# Autodesk Inventor assembly: PIVOT_FRAMING
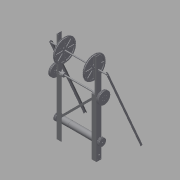
[picture p0: Inventor's stored thumbnail of the model, 180x180]
Saved by Autodesk Inventor 2014 SP1 (Build 180222100, 222)
## iProperties
Created: 2014-01-16
Part Number: PIVOT_FRAMING
Document SubType Name: Assembly
Designer: habib asif
Author: habib asif
## Documents named in this file (12)
- K:\MHS\Technology\Holliday B\Group Projects\Robotics\CAD Team\CAD Team 2014\shooter\Imported Components\top_level_ri3d\PIVOT_FRAMING.iam
- K:\MHS\Technology\Holliday B\Group Projects\Robotics\CAD Team\CAD Team 2014\shooter\Imported Components\top_level_ri3d\POST_PIVOT_FRAME.ipt
- K:\MHS\Technology\Holliday B\Group Projects\Robotics\CAD Team\CAD Team 2014\shooter\Imported Components\top_level_ri3d\PIVOT_POST_LEFT.ipt
- K:\MHS\Technology\Holliday B\Group Projects\Robotics\CAD Team\CAD Team 2014\shooter\Imported Components\top_level_ri3d\45_BRACE.ipt
- K:\MHS\Technology\Holliday B\Group Projects\Robotics\CAD Team\CAD Team 2014\shooter\Imported Components\top_level_ri3d\CIM_MOTOR.ipt
- K:\MHS\Technology\Holliday B\Group Projects\Robotics\CAD Team\CAD Team 2014\shooter\Imported Components\top_level_ri3d\MOTOR_PULLEY.ipt
- K:\MHS\Technology\Holliday B\Group Projects\Robotics\CAD Team\CAD Team 2014\shooter\Imported Components\top_level_ri3d\PULLEY2CHAIN.ipt
- K:\MHS\Technology\Holliday B\Group Projects\Robotics\CAD Team\CAD Team 2014\shooter\Imported Components\top_level_ri3d\TOP_SPROCKET_SHAFT.ipt
- K:\MHS\Technology\Holliday B\Group Projects\Robotics\CAD Team\CAD Team 2014\shooter\Imported Components\top_level_ri3d\CATAPULT_SUPPORT_LEFT.ipt
- K:\MHS\Technology\Holliday B\Group Projects\Robotics\CAD Team\CAD Team 2014\shooter\Imported Components\top_level_ri3d\CATAPULT_SUPPORT_RIGHT.ipt
- K:\MHS\Technology\Holliday B\Group Projects\Robotics\CAD Team\CAD Team 2014\shooter\Imported Components\top_level_ri3d\MOTOR_TUBING.ipt
- K:\MHS\Technology\Holliday B\Group Projects\Robotics\CAD Team\CAD Team 2014\shooter\Imported Components\top_level_ri3d\TOP_SPROCKET_ASM.iam
## Components (14 placed, 14 different names)
1. POST_PIVOT_FRAME_2 — Mate:1, Mate:2, Insert:1
2. PIVOT_POST_LEFT_3 — Mate:1, Mate:2, Insert:4
3. 45_BRACE_4
4. CIM_MOTOR_5 — Insert:8, Insert:9
5. CIM_MOTOR_6 — Insert:7, Insert:9
6. MOTOR_PULLEY_7 — Insert:7
7. PULLEY2CHAIN_8 — Insert:4
8. MOTOR_PULLEY_9 — Insert:8
9. TOP_SPROCKET_SHAFT_10 — Insert:1, Insert:2, Insert:3, Insert:5, Insert:6
10. CATAPULT_SUPPORT_LEFT_11 — Insert:6
11. CATAPULT_SUPPORT_RIGHT_12 — Insert:5
12. MOTOR_TUBING_13
13. TOP_SPROCKET_ASM_17 [sub-assembly] — Insert:3
14. TOP_SPROCKET_ASM_18 [sub-assembly] — Insert:2
## Relationships (11: Insert 9, Mate 2)
- Mate:1 (387.35 mm): POST_PIVOT_FRAME_2 ↔ PIVOT_POST_LEFT_3
- Mate:2 (387.35 mm): POST_PIVOT_FRAME_2 ↔ PIVOT_POST_LEFT_3
- Insert:1 (-101.6 mm): POST_PIVOT_FRAME_2 ↔ TOP_SPROCKET_SHAFT_10
- Insert:2 (-152.4 mm): TOP_SPROCKET_SHAFT_10 ↔ TOP_SPROCKET_ASM_18
- Insert:3 (-152.4 mm): TOP_SPROCKET_SHAFT_10 ↔ TOP_SPROCKET_ASM_17
- Insert:4 (12.7 mm): PIVOT_POST_LEFT_3 ↔ PULLEY2CHAIN_8
- Insert:5 (-117.475 mm): TOP_SPROCKET_SHAFT_10 ↔ CATAPULT_SUPPORT_RIGHT_12
- Insert:6 (-104.775 mm): TOP_SPROCKET_SHAFT_10 ↔ CATAPULT_SUPPORT_LEFT_11
- Insert:7 (-22.225 mm): CIM_MOTOR_6 ↔ MOTOR_PULLEY_7
- Insert:8 (-22.225 mm): CIM_MOTOR_5 ↔ MOTOR_PULLEY_9
- Insert:9 (-387.35 mm): CIM_MOTOR_5 ↔ CIM_MOTOR_6
